# Autodesk Inventor assembly: Y Carriage Assemby 1.0
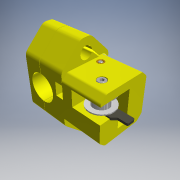
[picture p0: Inventor's stored thumbnail of the model, 180x180]
Saved by Autodesk Inventor 2016 (Build 200138000, 138)
## iProperties
Created: 2017-04-09
Part Number: Y Carriage Assemby 1.0
Document SubType Name: Assembly
Designer: Scott
Author: Scott
## Documents named in this file (10)
- E:\Scott Projects\3D Printing\CoreXY\Y Carriage Assemby 1.0.iam
- E:\Scott Projects\3D Printing\CoreXY\Y Carriage 1.0.ipt
- E:\Scott Projects\3D Printing\CoreXY\M3 Threaded Insert.ipt
- E:\Scott Projects\3D Printing\CoreXY\X End Stop Flag 1.0.ipt
- C:\Users\Scott\Documents\Inventor\Content Center Files\R2016\en-US\ANSI B18.3.1M(1)\ANSI B18.3.1M - M3x0.5 x 30(2).ipt
- E:\Scott Projects\3D Printing\CoreXY\GT2_20t_smooth_wheel_pulley.ipt
- E:\Scott Projects\3D Printing\CoreXY\GT2_20t_wheel_pulley.ipt
- C:\Users\Scott\Documents\Inventor\Content Center Files\R2016\en-US\ANSI B18.3.1M(1)\ANSI B18.3.1M - M3x0.5 x 16(2).ipt
- C:\Users\Scott\Documents\Inventor\Content Center Files\R2016\en-US\AS 1474(1)\AS 1474 - M3(1).ipt
- E:\Scott Projects\3D Printing\CoreXY\Y Carriage Clamp 1.0.ipt
## Components (21 placed, 9 different names)
1. Y Carriage 1.0:1 — Insert:1, Insert:2, Insert:3, Insert:4, Insert:5, Insert:6, Mate:1, Mate:2, Angle:1, Insert:7, Insert:8, Insert:9, Insert:10, Insert:11, Insert:12, Insert:13, Insert:14, Angle:2, Angle:3, Mate:3, Flush:1, Flush:2, Flush:3, Flush:4, Flush:5
2. M3 Threaded Insert:1 — Insert:1
3. M3 Threaded Insert:2 — Insert:4
4. M3 Threaded Insert:3 — Insert:3
5. M3 Threaded Insert:4 — Insert:2
6. M3 Threaded Insert:5 — Insert:5
7. M3 Threaded Insert:6 — Insert:6
8. X End Stop Flag 1.0:1 — Mate:1, Mate:2, Angle:1
9. Broached Socket Head Cap Screw - Metric M3x0.5 x 30:1 — Insert:7
10. Broached Socket Head Cap Screw - Metric M3x0.5 x 30:2 — Insert:8
11. GT2_20t_smooth_wheel_pulley:1 — Insert:9
12. GT2_20t_wheel_pulley:1 — Insert:10
13. Broached Socket Head Cap Screw - Metric M3x0.5 x 16:1 — Insert:11
14. Broached Socket Head Cap Screw - Metric M3x0.5 x 16:2 — Insert:12
15. AS 1474 - Metric M3:1 — Insert:13, Angle:3
16. AS 1474 - Metric M3:2 — Insert:14, Angle:2
17. Y Carriage Clamp 1.0:1 — Mate:3, Flush:1, Flush:2, Insert:15, Insert:16, Insert:17, Insert:18
18. Broached Socket Head Cap Screw - Metric M3x0.5 x 16:3 — Insert:15
19. Broached Socket Head Cap Screw - Metric M3x0.5 x 16:4 — Insert:18
20. Broached Socket Head Cap Screw - Metric M3x0.5 x 16:5 — Insert:17
21. Broached Socket Head Cap Screw - Metric M3x0.5 x 16:6 — Insert:16
## Relationships (29: Insert 18, Flush 5, Mate 3, Angle 3)
- Insert:1: Y Carriage 1.0:1 ↔ M3 Threaded Insert:1
- Insert:2: Y Carriage 1.0:1 ↔ M3 Threaded Insert:4
- Insert:3: Y Carriage 1.0:1 ↔ M3 Threaded Insert:3
- Insert:4: Y Carriage 1.0:1 ↔ M3 Threaded Insert:2
- Insert:5: Y Carriage 1.0:1 ↔ M3 Threaded Insert:5
- Insert:6: Y Carriage 1.0:1 ↔ M3 Threaded Insert:6
- Mate:1: Y Carriage 1.0:1 ↔ X End Stop Flag 1.0:1
- Mate:2: Y Carriage 1.0:1 ↔ X End Stop Flag 1.0:1
- Angle:1 (0 deg): Y Carriage 1.0:1 ↔ X End Stop Flag 1.0:1
- Insert:7: Y Carriage 1.0:1 ↔ Broached Socket Head Cap Screw - Metric M3x0.5 x 30:1
- Insert:8: Y Carriage 1.0:1 ↔ Broached Socket Head Cap Screw - Metric M3x0.5 x 30:2
- Insert:9: Y Carriage 1.0:1 ↔ GT2_20t_smooth_wheel_pulley:1
- Insert:10 (0.25 mm): Y Carriage 1.0:1 ↔ GT2_20t_wheel_pulley:1
- Insert:11: Y Carriage 1.0:1 ↔ Broached Socket Head Cap Screw - Metric M3x0.5 x 16:1
- Insert:12: Y Carriage 1.0:1 ↔ Broached Socket Head Cap Screw - Metric M3x0.5 x 16:2
- Insert:13: Y Carriage 1.0:1 ↔ AS 1474 - Metric M3:1
- Insert:14: Y Carriage 1.0:1 ↔ AS 1474 - Metric M3:2
- Angle:2 (0 deg): Y Carriage 1.0:1 ↔ AS 1474 - Metric M3:2
- Angle:3 (0 deg): Y Carriage 1.0:1 ↔ AS 1474 - Metric M3:1
- Mate:3 (0.25 mm): Y Carriage 1.0:1 ↔ Y Carriage Clamp 1.0:1
- Flush:1: Y Carriage 1.0:1 ↔ Y Carriage Clamp 1.0:1
- Flush:2: Y Carriage 1.0:1 ↔ Y Carriage Clamp 1.0:1
- Insert:15: Y Carriage Clamp 1.0:1 ↔ Broached Socket Head Cap Screw - Metric M3x0.5 x 16:3
- Flush:3: Y Carriage 1.0:1
- Flush:4: Y Carriage 1.0:1
- Flush:5: Y Carriage 1.0:1
- Insert:16: Y Carriage Clamp 1.0:1 ↔ Broached Socket Head Cap Screw - Metric M3x0.5 x 16:6
- Insert:17: Y Carriage Clamp 1.0:1 ↔ Broached Socket Head Cap Screw - Metric M3x0.5 x 16:5
- Insert:18: Y Carriage Clamp 1.0:1 ↔ Broached Socket Head Cap Screw - Metric M3x0.5 x 16:4
